# Autodesk Inventor assembly: UTM_Assembly
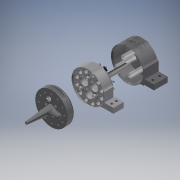
[picture p0: Inventor's stored thumbnail of the model, 180x180]
Saved by Autodesk Inventor 2017 (Build 210142000, 142)
## iProperties
Created: 2016-12-31
Part Number: UTM_Assembly
Document SubType Name: Assembly
Designer: umr
Author: umr
## Documents named in this file (13)
- D:\SeniorProject\Models2\UTM\UTM_Assembly.iam
- D:\SeniorProject\Models2\UTM\UTM Cover.ipt
- D:\SeniorProject\Models2\UTM\UTM.ipt
- D:\SeniorProject\Models2\UTM\12 wire cable.ipt
- D:\SeniorProject\Models2\UTM\1.5mm Square O-Ring 7.5mm ID (modelled as 8mm ID).ipt
- D:\SeniorProject\Models2\UTM\Grommet 9600k33.ipt
- D:\SeniorProject\Models2\UTM\Tubing.ipt
- D:\SeniorProject\Models2\UTM\M3 Screw_30mm.ipt
- D:\SeniorProject\Models2\UTM\M3 Spring 94125K472.ipt
- D:\SeniorProject\Models2\UTM\M3 Locknut.ipt
- D:\SeniorProject\Models2\UTM\Zip Tie.ipt
- D:\SeniorProject\Models2\UTM\MagnetAssembly.iam
- D:\SeniorProject\Models2\HeadTools\SeederAssembly.iam
## Components (21 placed, 12 different names)
1. UTM Cover:1 — Mate:1, Flush:1, Mate:2, Mate:6, Mate:7, Mate:8
2. UTM:1 — Mate:1, Flush:1, Mate:3, Mate:4, Mate:5, Mate:13, Mate:16, Mate:19, Mate:22, Mate:23, Mate:24, Mate:25, Mate:26, Mate:27, Mate:28
3. 12 wire cable:1 — Mate:2, Mate:9
4. 1.5mm Square O-Ring 7.5mm ID (modelled as 8mm ID):1 — Mate:5
5. 1.5mm Square O-Ring 7.5mm ID (modelled as 8mm ID):2 — Mate:4
6. 1.5mm Square O-Ring 7.5mm ID (modelled as 8mm ID):3 — Mate:3
7. Grommet 9600k33:1 — Mate:9
8. Grommet 9600k33:2 — Mate:10
9. Grommet 9600k33:3 — Mate:12
10. Grommet 9600k33:4 — Mate:11
11. Tubing:1 — Mate:8, Mate:12
12. Tubing:2 — Mate:7, Mate:11
13. Tubing:3 — Mate:6, Mate:10
14. M3 Spring 94125K472:1 — Mate:15, Mate:16, Mate:17
15. M3 Locknut:1 — Mate:18, Mate:19, Mate:21
16. M3 Screw_30mm:1 — Mate:13, Mate:15, Mate:17, Mate:18, Mate:20
17. Zip Tie:1 — Mate:20, Mate:21
18. MagnetAssembly:1 [sub-assembly] — Mate:22, Mate:27
19. MagnetAssembly:2 [sub-assembly] — Mate:23, Mate:26
20. MagnetAssembly:3 [sub-assembly] — Mate:24, Mate:25
21. SeederAssembly:1 [sub-assembly] — Mate:28
## Relationships (28: Mate 27, Flush 1)
- Mate:1: UTM Cover:1 ↔ UTM:1
- Flush:1: UTM Cover:1 ↔ UTM:1
- Mate:2: UTM Cover:1 ↔ 12 wire cable:1
- Mate:3: UTM:1 ↔ 1.5mm Square O-Ring 7.5mm ID (modelled as 8mm ID):3
- Mate:4: UTM:1 ↔ 1.5mm Square O-Ring 7.5mm ID (modelled as 8mm ID):2
- Mate:5: UTM:1 ↔ 1.5mm Square O-Ring 7.5mm ID (modelled as 8mm ID):1
- Mate:6: UTM Cover:1 ↔ Tubing:3
- Mate:7: UTM Cover:1 ↔ Tubing:2
- Mate:8: UTM Cover:1 ↔ Tubing:1
- Mate:9: 12 wire cable:1 ↔ Grommet 9600k33:1
- Mate:10: Grommet 9600k33:2 ↔ Tubing:3
- Mate:11: Grommet 9600k33:4 ↔ Tubing:2
- Mate:12: Grommet 9600k33:3 ↔ Tubing:1
- Mate:13: UTM:1 ↔ M3 Screw_30mm:1
- Mate:15: M3 Spring 94125K472:1 ↔ M3 Screw_30mm:1
- Mate:16: UTM:1 ↔ M3 Spring 94125K472:1
- Mate:17: M3 Spring 94125K472:1 ↔ M3 Screw_30mm:1
- Mate:18: M3 Locknut:1 ↔ M3 Screw_30mm:1
- Mate:19: UTM:1 ↔ M3 Locknut:1
- Mate:20: M3 Screw_30mm:1 ↔ Zip Tie:1
- Mate:21: M3 Locknut:1 ↔ Zip Tie:1
- Mate:22: UTM:1 ↔ MagnetAssembly:1
- Mate:23: UTM:1 ↔ MagnetAssembly:2
- Mate:24: UTM:1 ↔ MagnetAssembly:3
- Mate:25: UTM:1 ↔ MagnetAssembly:3
- Mate:26: UTM:1 ↔ MagnetAssembly:2
- Mate:27: UTM:1 ↔ MagnetAssembly:1
- Mate:28: UTM:1 ↔ SeederAssembly:1
